(part 1 of 2)
# Autodesk Inventor assembly: 110033226_iam_04_大橋塔樓
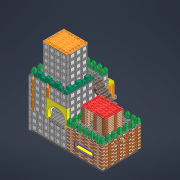
[picture p0: Inventor's stored thumbnail of the model, 180x180]
Saved by Autodesk Inventor 2022 (Build 260153000, 153)
## iProperties
Created: 2022-06-23
Part Number: 110033226_iam_04_大橋塔樓
Document SubType Name: Assembly
Designer: User
Author: User
## Documents named in this file (16)
- D:\D-disk\pomelo\大一\下學期\機械設計製圖\1100332260_LEGOproj_沒有公主城堡\110033226_iam_04_大橋塔樓.iam
- D:\D-disk\pomelo\大一\下學期\機械設計製圖\1100332260_LEGOproj_沒有公主城堡\110033226_ipt_07_磚塊樺木(2x1).ipt
- D:\D-disk\pomelo\大一\下學期\機械設計製圖\1100332260_LEGOproj_沒有公主城堡\110033226_ipt_05_房子底座.ipt
- D:\D-disk\pomelo\大一\下學期\機械設計製圖\1100332260_LEGOproj_沒有公主城堡\110033226_ipt_06_磚塊樺木(1x1).ipt
- D:\D-disk\pomelo\大一\下學期\機械設計製圖\1100332260_LEGOproj_沒有公主城堡\110033226_ipt_16_圍牆.ipt
- D:\D-disk\pomelo\大一\下學期\機械設計製圖\1100332260_LEGOproj_沒有公主城堡\110033226_ipt_08_平滑面(3x1).ipt
- D:\D-disk\pomelo\大一\下學期\機械設計製圖\1100332260_LEGOproj_沒有公主城堡\110033226_ipt_20_塔樓窗戶.ipt
- D:\D-disk\pomelo\大一\下學期\機械設計製圖\1100332260_LEGOproj_沒有公主城堡\110033226_ipt_21_柵欄.ipt
- D:\D-disk\pomelo\大一\下學期\機械設計製圖\1100332260_LEGOproj_沒有公主城堡\110033226_ipt_11_樓梯支架.ipt
- D:\D-disk\pomelo\大一\下學期\機械設計製圖\1100332260_LEGOproj_沒有公主城堡\110033226_ipt_22_塔樓牆壁.ipt
- D:\D-disk\pomelo\大一\下學期\機械設計製圖\1100332260_LEGOproj_沒有公主城堡\110033226_ipt_23_塔樓門口.ipt
- D:\D-disk\pomelo\大一\下學期\機械設計製圖\1100332260_LEGOproj_沒有公主城堡\110033226_ipt_10_木板條.ipt
- D:\D-disk\pomelo\大一\下學期\機械設計製圖\1100332260_LEGOproj_沒有公主城堡\110033226_ipt_24_直條(3x1).ipt
- D:\D-disk\pomelo\大一\下學期\機械設計製圖\1100332260_LEGOproj_沒有公主城堡\110033226_ipt_25_塔樓大窗戶.ipt
- D:\D-disk\pomelo\大一\下學期\機械設計製圖\1100332260_LEGOproj_沒有公主城堡\110033226_ipt_12_平滑面(2x1).ipt
- D:\D-disk\pomelo\大一\下學期\機械設計製圖\1100332260_LEGOproj_沒有公主城堡\110033226_ipt_18_大橋圍牆.ipt
## Components (1151 placed, 15 different names)
1. 110033226_ipt_05_房子底座:1 — 貼合:1, 貼合:2, 貼合:3, 貼合:4, 貼合:5, 貼合:13, 貼合:14, 貼合:15, 貼合:16, 貼合:17, 貼合:96, 貼合:97
2. 110033226_ipt_07_磚塊樺木(2x1):1 — 貼合:28, 貼合:29, 貼合:30, 貼合:148
3. 110033226_ipt_20_塔樓窗戶:1 — 貼合:37, 貼合:38, 貼合:39, 貼合:40
4. 110033226_ipt_20_塔樓窗戶:2 — 貼合:41, 貼合:42, 貼合:43
5. 110033226_ipt_08_平滑面(3x1):58 — 貼合:69, 貼合:70, 貼合:71, 貼合:193, 貼合:194, 貼合:195, 貼合:202, 貼合:204
6. 110033226_ipt_08_平滑面(3x1):59 — 貼合:72, 貼合:73, 貼合:74
7. 110033226_ipt_08_平滑面(3x1):60 — 貼合:75, 貼合:82, 貼合:83
8. 110033226_ipt_08_平滑面(3x1):61 — 貼合:76, 貼合:84, 貼合:85
9. 110033226_ipt_08_平滑面(3x1):62 — 貼合:78, 貼合:86, 貼合:87
10. 110033226_ipt_08_平滑面(3x1):63 — 貼合:80, 貼合:94, 貼合:95
11. 110033226_ipt_08_平滑面(3x1):64 — 貼合:77, 貼合:88, 貼合:89
12. 110033226_ipt_08_平滑面(3x1):65 — 貼合:79, 貼合:90, 貼合:91
13. 110033226_ipt_08_平滑面(3x1):66 — 貼合:81, 貼合:92, 貼合:93
14. 110033226_ipt_05_房子底座:2 — 貼合:96, 貼合:97, 貼合:98, 貼合:99, 貼合:100, 貼合:101, 對稱:1, 貼合:102, 貼合:103, 貼合:137, 貼合:138, 貼合:139, 貼合:143, 貼合:144, 貼合:145, 貼合:146, 貼合:147, 貼合:170
15. 110033226_ipt_23_塔樓門口:1 — 貼合:104, 貼合:105, 貼合:106, 貼合:179, 貼合:180, 貼合:181, 貼合:182, 貼合:183
16. 110033226_ipt_10_木板條:1 — 貼合:134, 貼合:135, 貼合:136
17. 110033226_ipt_10_木板條:33 — 貼合:128, 貼合:129, 貼合:130
18. 110033226_ipt_10_木板條:34 — 貼合:113, 貼合:114, 貼合:115, 貼合:116, 貼合:117, 貼合:118
19. 110033226_ipt_10_木板條:35 — 貼合:140, 貼合:141, 貼合:142
20. 110033226_ipt_10_木板條:36 — 貼合:131, 貼合:132, 貼合:133
21. 110033226_ipt_10_木板條:42 — 貼合:119, 貼合:120, 貼合:121
22. 110033226_ipt_24_直條(3x1):8 — 貼合:182, 貼合:183
23. 110033226_ipt_25_塔樓大窗戶:1 — 貼合:196, 貼合:197, 貼合:198
24. 110033226_ipt_16_圍牆:1 — 貼合:25, 貼合:26, 貼合:27
25. 110033226_ipt_16_圍牆:2
26. 110033226_ipt_21_柵欄:1 — 貼合:44, 貼合:45, 貼合:46, 貼合:48
27. 110033226_ipt_21_柵欄:4
28. 110033226_ipt_21_柵欄:5
29. 110033226_ipt_21_柵欄:6
30. 110033226_ipt_21_柵欄:7
31. 110033226_ipt_21_柵欄:8
32. 110033226_ipt_21_柵欄:9
33. 110033226_ipt_21_柵欄:14
34. 110033226_ipt_21_柵欄:15
35. 110033226_ipt_21_柵欄:16
36. 110033226_ipt_21_柵欄:17
37. 110033226_ipt_21_柵欄:18
38. 110033226_ipt_21_柵欄:19
39. 110033226_ipt_21_柵欄:20
40. 110033226_ipt_21_柵欄:2 — 貼合:47, 貼合:48, 貼合:49
41. 110033226_ipt_21_柵欄:10
42. 110033226_ipt_21_柵欄:11
43. 110033226_ipt_21_柵欄:12
44. 110033226_ipt_21_柵欄:13
45. 110033226_ipt_21_柵欄:21
46. 110033226_ipt_21_柵欄:22
47. 110033226_ipt_21_柵欄:23
48. 110033226_ipt_21_柵欄:24
49. 110033226_ipt_21_柵欄:25
50. 110033226_ipt_22_塔樓牆壁:2 — 對稱:1, 貼合:102, 貼合:103
51. 110033226_ipt_22_塔樓牆壁:22
52. 110033226_ipt_22_塔樓牆壁:23
53. 110033226_ipt_22_塔樓牆壁:24
54. 110033226_ipt_22_塔樓牆壁:25
55. 110033226_ipt_22_塔樓牆壁:26
56. 110033226_ipt_22_塔樓牆壁:27
57. 110033226_ipt_22_塔樓牆壁:28
58. 110033226_ipt_22_塔樓牆壁:29
59. 110033226_ipt_22_塔樓牆壁:30
60. 110033226_ipt_22_塔樓牆壁:31
61. 110033226_ipt_22_塔樓牆壁:32
62. 110033226_ipt_22_塔樓牆壁:33
63. 110033226_ipt_22_塔樓牆壁:34
64. 110033226_ipt_22_塔樓牆壁:35
65. 110033226_ipt_22_塔樓牆壁:36
66. 110033226_ipt_22_塔樓牆壁:37
67. 110033226_ipt_22_塔樓牆壁:38
68. 110033226_ipt_22_塔樓牆壁:39
69. 110033226_ipt_22_塔樓牆壁:40
70. 110033226_ipt_22_塔樓牆壁:41 — 貼合:171, 貼合:172
71. 110033226_ipt_22_塔樓牆壁:42
72. 110033226_ipt_22_塔樓牆壁:43
73. 110033226_ipt_22_塔樓牆壁:44
74. 110033226_ipt_22_塔樓牆壁:45 — 貼合:173, 貼合:174, 貼合:175
75. 110033226_ipt_22_塔樓牆壁:46 — 貼合:107, 貼合:108, 貼合:109
76. 110033226_ipt_22_塔樓牆壁:48
77. 110033226_ipt_22_塔樓牆壁:49
78. 110033226_ipt_22_塔樓牆壁:50
79. 110033226_ipt_22_塔樓牆壁:51 — 貼合:215
80. 110033226_ipt_22_塔樓牆壁:52
81. 110033226_ipt_22_塔樓牆壁:53
82. 110033226_ipt_22_塔樓牆壁:54
83. 110033226_ipt_22_塔樓牆壁:215
84. 110033226_ipt_22_塔樓牆壁:216 — 貼合:213, 貼合:214
85. 110033226_ipt_11_樓梯支架:41 — 貼合:113, 貼合:114, 貼合:118, 貼合:119, 貼合:121
86. 110033226_ipt_11_樓梯支架:42 — 貼合:120
87. 110033226_ipt_11_樓梯支架:43 — 貼合:134
88. 110033226_ipt_11_樓梯支架:44 — 貼合:135, 貼合:136
89. 110033226_ipt_11_樓梯支架:45 — 貼合:123
90. 110033226_ipt_11_樓梯支架:46 — 貼合:122, 貼合:124
91. 110033226_ipt_10_木板條:3 — 貼合:122, 貼合:123, 貼合:124
92. 110033226_ipt_10_木板條:43
93. 110033226_ipt_10_木板條:44 — 貼合:125, 貼合:126, 貼合:127
94. 110033226_ipt_11_樓梯支架:40 — 貼合:125, 貼合:126, 貼合:127, 貼合:142
95. 110033226_ipt_11_樓梯支架:47 — 貼合:140, 貼合:141
96. 110033226_ipt_11_樓梯支架:48 — 貼合:131, 貼合:133
97. 110033226_ipt_11_樓梯支架:49 — 貼合:132
98. 110033226_ipt_11_樓梯支架:50 — 貼合:129
99. 110033226_ipt_11_樓梯支架:51 — 貼合:128, 貼合:130
100. 110033226_ipt_10_木板條:39 — 貼合:137, 貼合:138, 貼合:139
101. 110033226_ipt_10_木板條:45
102. 110033226_ipt_22_塔樓牆壁:55 — 貼合:143, 貼合:144, 貼合:145, 對稱:2, 貼合:152, 貼合:153
103. 110033226_ipt_22_塔樓牆壁:140
104. 110033226_ipt_22_塔樓牆壁:141
105. 110033226_ipt_22_塔樓牆壁:142 — 貼合:196
106. 110033226_ipt_22_塔樓牆壁:143
107. 110033226_ipt_22_塔樓牆壁:144
108. 110033226_ipt_22_塔樓牆壁:145 — 貼合:149, 貼合:150, 貼合:151
109. 110033226_ipt_22_塔樓牆壁:147 — 貼合:149, 貼合:150, 貼合:151, 貼合:198
110. 110033226_ipt_22_塔樓牆壁:149
111. 110033226_ipt_22_塔樓牆壁:148 — 對稱:2, 貼合:152, 貼合:153
112. 110033226_ipt_22_塔樓牆壁:150
113. 110033226_ipt_22_塔樓牆壁:151 — 貼合:178
114. 110033226_ipt_22_塔樓牆壁:152
115. 110033226_ipt_22_塔樓牆壁:153
116. 110033226_ipt_22_塔樓牆壁:154
117. 110033226_ipt_22_塔樓牆壁:155
118. 110033226_ipt_22_塔樓牆壁:156
119. 110033226_ipt_22_塔樓牆壁:157
120. 110033226_ipt_22_塔樓牆壁:158 — 貼合:197
121. 110033226_ipt_22_塔樓牆壁:159
122. 110033226_ipt_22_塔樓牆壁:160
123. 110033226_ipt_22_塔樓牆壁:161 — 貼合:199, 貼合:200, 貼合:201
124. 110033226_ipt_22_塔樓牆壁:162 — 貼合:205
125. 110033226_ipt_07_磚塊樺木(2x1):234 — 對稱:3, 貼合:163, 貼合:164, 貼合:165, 貼合:166, 貼合:167
126. 110033226_ipt_06_磚塊樺木(1x1):234 — 貼合:165, 貼合:166, 貼合:167
127. 110033226_ipt_07_磚塊樺木(2x1):235
128. 110033226_ipt_06_磚塊樺木(1x1):235
129. 110033226_ipt_07_磚塊樺木(2x1):236
130. 110033226_ipt_06_磚塊樺木(1x1):236
131. 110033226_ipt_07_磚塊樺木(2x1):237
132. 110033226_ipt_06_磚塊樺木(1x1):237
133. 110033226_ipt_07_磚塊樺木(2x1):238
134. 110033226_ipt_06_磚塊樺木(1x1):238
135. 110033226_ipt_07_磚塊樺木(2x1):239
136. 110033226_ipt_06_磚塊樺木(1x1):239
137. 110033226_ipt_07_磚塊樺木(2x1):240
138. 110033226_ipt_06_磚塊樺木(1x1):240
139. 110033226_ipt_07_磚塊樺木(2x1):241
140. 110033226_ipt_06_磚塊樺木(1x1):241
141. 110033226_ipt_07_磚塊樺木(2x1):242
142. 110033226_ipt_06_磚塊樺木(1x1):242
143. 110033226_ipt_07_磚塊樺木(2x1):243
144. 110033226_ipt_06_磚塊樺木(1x1):243
145. 110033226_ipt_07_磚塊樺木(2x1):244
146. 110033226_ipt_06_磚塊樺木(1x1):244
147. 110033226_ipt_07_磚塊樺木(2x1):245
148. 110033226_ipt_06_磚塊樺木(1x1):245
149. 110033226_ipt_07_磚塊樺木(2x1):246
150. 110033226_ipt_06_磚塊樺木(1x1):246
151. 110033226_ipt_07_磚塊樺木(2x1):247
152. 110033226_ipt_06_磚塊樺木(1x1):247
153. 110033226_ipt_07_磚塊樺木(2x1):248
154. 110033226_ipt_06_磚塊樺木(1x1):248
155. 110033226_ipt_07_磚塊樺木(2x1):249
156. 110033226_ipt_06_磚塊樺木(1x1):249
157. 110033226_ipt_07_磚塊樺木(2x1):250
158. 110033226_ipt_06_磚塊樺木(1x1):250
159. 110033226_ipt_07_磚塊樺木(2x1):251
160. 110033226_ipt_06_磚塊樺木(1x1):251
161. 110033226_ipt_07_磚塊樺木(2x1):252
162. 110033226_ipt_06_磚塊樺木(1x1):252
163. 110033226_ipt_07_磚塊樺木(2x1):253
164. 110033226_ipt_06_磚塊樺木(1x1):253
165. 110033226_ipt_07_磚塊樺木(2x1):228 — 貼合:57, 貼合:58, 貼合:59, 貼合:61, 貼合:62
166. 110033226_ipt_06_磚塊樺木(1x1):229 — 貼合:60, 貼合:61, 貼合:62
167. 110033226_ipt_07_磚塊樺木(2x1):254
168. 110033226_ipt_06_磚塊樺木(1x1):254
169. 110033226_ipt_07_磚塊樺木(2x1):259
170. 110033226_ipt_06_磚塊樺木(1x1):259
171. 110033226_ipt_07_磚塊樺木(2x1):264
172. 110033226_ipt_06_磚塊樺木(1x1):264
173. 110033226_ipt_07_磚塊樺木(2x1):269
174. 110033226_ipt_06_磚塊樺木(1x1):269
175. 110033226_ipt_07_磚塊樺木(2x1):274
176. 110033226_ipt_06_磚塊樺木(1x1):274
177. 110033226_ipt_07_磚塊樺木(2x1):279
178. 110033226_ipt_06_磚塊樺木(1x1):279
179. 110033226_ipt_07_磚塊樺木(2x1):284
180. 110033226_ipt_06_磚塊樺木(1x1):284
181. 110033226_ipt_07_磚塊樺木(2x1):289
182. 110033226_ipt_06_磚塊樺木(1x1):289
183. 110033226_ipt_07_磚塊樺木(2x1):294
184. 110033226_ipt_06_磚塊樺木(1x1):294 — 貼合:245
185. 110033226_ipt_06_磚塊樺木(1x1):299 — 對稱:4, 貼合:168, 貼合:169
186. 110033226_ipt_06_磚塊樺木(1x1):300
187. 110033226_ipt_06_磚塊樺木(1x1):301
188. 110033226_ipt_06_磚塊樺木(1x1):302
189. 110033226_ipt_06_磚塊樺木(1x1):303
190. 110033226_ipt_06_磚塊樺木(1x1):304
191. 110033226_ipt_06_磚塊樺木(1x1):305
192. 110033226_ipt_06_磚塊樺木(1x1):306
193. 110033226_ipt_06_磚塊樺木(1x1):307
194. 110033226_ipt_06_磚塊樺木(1x1):308 — 貼合:241, 貼合:242, 貼合:243, 貼合:244
195. 110033226_ipt_24_直條(3x1):1 — 貼合:170, 貼合:171, 貼合:172
196. 110033226_ipt_24_直條(3x1):2
197. 110033226_ipt_24_直條(3x1):3
198. 110033226_ipt_24_直條(3x1):4
199. 110033226_ipt_22_塔樓牆壁:194 — 貼合:173, 貼合:174, 貼合:175
200. 110033226_ipt_22_塔樓牆壁:206
201. 110033226_ipt_22_塔樓牆壁:207
202. 110033226_ipt_22_塔樓牆壁:208 — 貼合:184
203. 110033226_ipt_22_塔樓牆壁:209 — 貼合:185, 貼合:186
204. 110033226_ipt_24_直條(3x1):5 — 貼合:176, 貼合:177, 貼合:178
205. 110033226_ipt_24_直條(3x1):6
206. 110033226_ipt_24_直條(3x1):7
207. 110033226_ipt_22_塔樓牆壁:193 — 貼合:179, 貼合:180, 貼合:181
208. 110033226_ipt_22_塔樓牆壁:210
209. 110033226_ipt_22_塔樓牆壁:211
210. 110033226_ipt_22_塔樓牆壁:212
211. 110033226_ipt_22_塔樓牆壁:213
212. 110033226_ipt_22_塔樓牆壁:214
213. 110033226_ipt_22_塔樓牆壁:217 — 貼合:184, 貼合:185, 貼合:186
214. 110033226_ipt_22_塔樓牆壁:218
215. 110033226_ipt_22_塔樓牆壁:219
216. 110033226_ipt_22_塔樓牆壁:220
217. 110033226_ipt_22_塔樓牆壁:221
218. 110033226_ipt_22_塔樓牆壁:222 — 貼合:218
219. 110033226_ipt_22_塔樓牆壁:223
220. 110033226_ipt_22_塔樓牆壁:224 — 貼合:216, 貼合:217
221. 110033226_ipt_22_塔樓牆壁:225 — 貼合:187, 貼合:188, 貼合:189
222. 110033226_ipt_22_塔樓牆壁:226 — 貼合:190, 貼合:191, 貼合:192
223. 110033226_ipt_21_柵欄:26 — 貼合:190, 貼合:191, 貼合:192
224. 110033226_ipt_21_柵欄:27
225. 110033226_ipt_21_柵欄:28
226. 110033226_ipt_21_柵欄:29
227. 110033226_ipt_21_柵欄:30
228. 110033226_ipt_21_柵欄:31
229. 110033226_ipt_21_柵欄:32
230. 110033226_ipt_21_柵欄:33
231. 110033226_ipt_21_柵欄:34
232. 110033226_ipt_21_柵欄:35
233. 110033226_ipt_21_柵欄:36
234. 110033226_ipt_21_柵欄:37
235. 110033226_ipt_08_平滑面(3x1):67 — 貼合:193, 貼合:194, 貼合:195
236. 110033226_ipt_08_平滑面(3x1):70 — 貼合:203
237. 110033226_ipt_08_平滑面(3x1):71 — 貼合:208, 貼合:222, 貼合:223, 貼合:224
238. 110033226_ipt_08_平滑面(3x1):72
239. 110033226_ipt_08_平滑面(3x1):73 — 貼合:225, 貼合:226
240. 110033226_ipt_08_平滑面(3x1):74
241. 110033226_ipt_08_平滑面(3x1):75
242. 110033226_ipt_08_平滑面(3x1):76 — 貼合:227
243. 110033226_ipt_08_平滑面(3x1):77
244. 110033226_ipt_08_平滑面(3x1):78
245. 110033226_ipt_08_平滑面(3x1):79
246. 110033226_ipt_08_平滑面(3x1):80
247. 110033226_ipt_08_平滑面(3x1):81
248. 110033226_ipt_08_平滑面(3x1):82
249. 110033226_ipt_08_平滑面(3x1):83
250. 110033226_ipt_08_平滑面(3x1):84
251. 110033226_ipt_08_平滑面(3x1):85
252. 110033226_ipt_08_平滑面(3x1):86
253. 110033226_ipt_08_平滑面(3x1):87
254. 110033226_ipt_08_平滑面(3x1):88
255. 110033226_ipt_08_平滑面(3x1):89
256. 110033226_ipt_08_平滑面(3x1):90
257. 110033226_ipt_08_平滑面(3x1):91 — 貼合:228, 貼合:229, 貼合:230
258. 110033226_ipt_08_平滑面(3x1):92
259. 110033226_ipt_08_平滑面(3x1):93
260. 110033226_ipt_08_平滑面(3x1):94
261. 110033226_ipt_08_平滑面(3x1):95 — 貼合:206
262. 110033226_ipt_08_平滑面(3x1):96
263. 110033226_ipt_08_平滑面(3x1):97
264. 110033226_ipt_08_平滑面(3x1):98 — 貼合:207
265. 110033226_ipt_22_塔樓牆壁:227 — 貼合:199, 貼合:200, 貼合:201
266. 110033226_ipt_22_塔樓牆壁:229
267. 110033226_ipt_22_塔樓牆壁:230
268. 110033226_ipt_22_塔樓牆壁:231
269. 110033226_ipt_22_塔樓牆壁:232
270. 110033226_ipt_22_塔樓牆壁:233
271. 110033226_ipt_22_塔樓牆壁:234
272. 110033226_ipt_22_塔樓牆壁:235 — 貼合:211, 貼合:212
273. 110033226_ipt_08_平滑面(3x1):100 — 貼合:202, 貼合:203, 貼合:204
274. 110033226_ipt_08_平滑面(3x1):102 — 貼合:210
275. 110033226_ipt_08_平滑面(3x1):101 — 貼合:205, 貼合:206, 貼合:207
276. 110033226_ipt_08_平滑面(3x1):103
277. 110033226_ipt_08_平滑面(3x1):104 — 貼合:209, 貼合:220
278. 110033226_ipt_08_平滑面(3x1):105
279. 110033226_ipt_08_平滑面(3x1):106
280. 110033226_ipt_08_平滑面(3x1):107
281. 110033226_ipt_12_平滑面(2x1):1 — 貼合:208, 貼合:209, 貼合:210, 貼合:219, 貼合:221
282. 110033226_ipt_12_平滑面(2x1):3
283. 110033226_ipt_21_柵欄:42 — 貼合:211, 貼合:212
284. 110033226_ipt_21_柵欄:43
285. 110033226_ipt_21_柵欄:44
286. 110033226_ipt_21_柵欄:45
287. 110033226_ipt_21_柵欄:46
288. 110033226_ipt_21_柵欄:47
289. 110033226_ipt_21_柵欄:48
290. 110033226_ipt_21_柵欄:49
291. 110033226_ipt_21_柵欄:50
292. 110033226_ipt_21_柵欄:51
293. 110033226_ipt_21_柵欄:52
294. 110033226_ipt_21_柵欄:53
295. 110033226_ipt_18_大橋圍牆:2 — 貼合:213, 貼合:214, 貼合:215
296. 110033226_ipt_18_大橋圍牆:3
297. 110033226_ipt_18_大橋圍牆:4
298. 110033226_ipt_18_大橋圍牆:1 — 貼合:216, 貼合:217, 貼合:218
299. 110033226_ipt_18_大橋圍牆:5
300. 110033226_ipt_18_大橋圍牆:6
301. 110033226_ipt_12_平滑面(2x1):4 — 貼合:234, 貼合:235, 貼合:236
302. 110033226_ipt_12_平滑面(2x1):8
303. 110033226_ipt_12_平滑面(2x1):9
304. 110033226_ipt_12_平滑面(2x1):10
305. 110033226_ipt_12_平滑面(2x1):11
306. 110033226_ipt_12_平滑面(2x1):12
307. 110033226_ipt_12_平滑面(2x1):13
308. 110033226_ipt_12_平滑面(2x1):14
309. 110033226_ipt_12_平滑面(2x1):15
310. 110033226_ipt_12_平滑面(2x1):16
311. 110033226_ipt_12_平滑面(2x1):17
312. 110033226_ipt_12_平滑面(2x1):18
313. 110033226_ipt_12_平滑面(2x1):19
314. 110033226_ipt_12_平滑面(2x1):20
315. 110033226_ipt_12_平滑面(2x1):21
316. 110033226_ipt_12_平滑面(2x1):22
317. 110033226_ipt_12_平滑面(2x1):23
318. 110033226_ipt_12_平滑面(2x1):24
319. 110033226_ipt_12_平滑面(2x1):25
320. 110033226_ipt_12_平滑面(2x1):26
321. 110033226_ipt_12_平滑面(2x1):27
322. 110033226_ipt_12_平滑面(2x1):28
323. 110033226_ipt_12_平滑面(2x1):29
324. 110033226_ipt_12_平滑面(2x1):30
325. 110033226_ipt_12_平滑面(2x1):31
326. 110033226_ipt_12_平滑面(2x1):32
327. 110033226_ipt_12_平滑面(2x1):33
328. 110033226_ipt_12_平滑面(2x1):34
329. 110033226_ipt_22_塔樓牆壁:298 — 貼合:237, 貼合:238, 貼合:239
330. 110033226_ipt_22_塔樓牆壁:299
331. 110033226_ipt_22_塔樓牆壁:300
332. 110033226_ipt_12_平滑面(2x1):35
333. 110033226_ipt_12_平滑面(2x1):36
334. 110033226_ipt_12_平滑面(2x1):37
335. 110033226_ipt_12_平滑面(2x1):38
336. 110033226_ipt_12_平滑面(2x1):39
337. 110033226_ipt_12_平滑面(2x1):40
338. 110033226_ipt_12_平滑面(2x1):41
339. 110033226_ipt_12_平滑面(2x1):42
340. 110033226_ipt_12_平滑面(2x1):43
341. 110033226_ipt_12_平滑面(2x1):44
342. 110033226_ipt_12_平滑面(2x1):45
343. 110033226_ipt_12_平滑面(2x1):46
344. 110033226_ipt_12_平滑面(2x1):47
345. 110033226_ipt_12_平滑面(2x1):48
346. 110033226_ipt_08_平滑面(3x1):110 — 貼合:240, 貼合:241, 貼合:242
347. 110033226_ipt_08_平滑面(3x1):111
348. 110033226_ipt_08_平滑面(3x1):112
349. 110033226_ipt_08_平滑面(3x1):113
350. 110033226_ipt_08_平滑面(3x1):108 — 貼合:243, 貼合:244, 貼合:245
351. 110033226_ipt_08_平滑面(3x1):114
352. 110033226_ipt_08_平滑面(3x1):115
353. 110033226_ipt_08_平滑面(3x1):116
354. 110033226_ipt_08_平滑面(3x1):117
355. 110033226_ipt_08_平滑面(3x1):118
356. 110033226_ipt_08_平滑面(3x1):119
357. 110033226_ipt_08_平滑面(3x1):120
358. 110033226_ipt_08_平滑面(3x1):121
359. 110033226_ipt_08_平滑面(3x1):122
360. 110033226_ipt_08_平滑面(3x1):123
361. 110033226_ipt_08_平滑面(3x1):124
362. 110033226_ipt_06_磚塊樺木(1x1):2 — 貼合:22, 貼合:23, 貼合:24
363. 110033226_ipt_07_磚塊樺木(2x1):2 — 貼合:19, 貼合:20, 貼合:21, 貼合:23
364. 110033226_ipt_06_磚塊樺木(1x1):1 — 貼合:16, 貼合:17, 貼合:18, 貼合:19, 貼合:21
365. 110033226_ipt_07_磚塊樺木(2x1):5 — 貼合:13, 貼合:14, 貼合:15, 貼合:18, 貼合:20, 貼合:22, 貼合:24
366. 110033226_ipt_06_磚塊樺木(1x1):60
367. 110033226_ipt_07_磚塊樺木(2x1):61
368. 110033226_ipt_06_磚塊樺木(1x1):61
369. 110033226_ipt_07_磚塊樺木(2x1):62
370. 110033226_ipt_06_磚塊樺木(1x1):62
371. 110033226_ipt_07_磚塊樺木(2x1):63
372. 110033226_ipt_06_磚塊樺木(1x1):63
373. 110033226_ipt_07_磚塊樺木(2x1):64
374. 110033226_ipt_06_磚塊樺木(1x1):64
375. 110033226_ipt_07_磚塊樺木(2x1):65
376. 110033226_ipt_06_磚塊樺木(1x1):65
377. 110033226_ipt_07_磚塊樺木(2x1):66
378. 110033226_ipt_06_磚塊樺木(1x1):66
379. 110033226_ipt_07_磚塊樺木(2x1):67
380. 110033226_ipt_06_磚塊樺木(1x1):67
381. 110033226_ipt_07_磚塊樺木(2x1):68
382. 110033226_ipt_06_磚塊樺木(1x1):68
383. 110033226_ipt_07_磚塊樺木(2x1):69
384. 110033226_ipt_06_磚塊樺木(1x1):69
385. 110033226_ipt_07_磚塊樺木(2x1):70
386. 110033226_ipt_06_磚塊樺木(1x1):70
387. 110033226_ipt_07_磚塊樺木(2x1):71
388. 110033226_ipt_06_磚塊樺木(1x1):71
389. 110033226_ipt_07_磚塊樺木(2x1):72
390. 110033226_ipt_06_磚塊樺木(1x1):72
391. 110033226_ipt_07_磚塊樺木(2x1):73
392. 110033226_ipt_06_磚塊樺木(1x1):73
393. 110033226_ipt_07_磚塊樺木(2x1):74
394. 110033226_ipt_06_磚塊樺木(1x1):74
395. 110033226_ipt_07_磚塊樺木(2x1):75
396. 110033226_ipt_06_磚塊樺木(1x1):75
397. 110033226_ipt_07_磚塊樺木(2x1):76
398. 110033226_ipt_06_磚塊樺木(1x1):76
399. 110033226_ipt_07_磚塊樺木(2x1):77
400. 110033226_ipt_06_磚塊樺木(1x1):77
401. 110033226_ipt_07_磚塊樺木(2x1):78
402. 110033226_ipt_06_磚塊樺木(1x1):78
403. 110033226_ipt_07_磚塊樺木(2x1):79
404. 110033226_ipt_06_磚塊樺木(1x1):79
405. 110033226_ipt_07_磚塊樺木(2x1):80
406. 110033226_ipt_06_磚塊樺木(1x1):80
407. 110033226_ipt_07_磚塊樺木(2x1):81
408. 110033226_ipt_06_磚塊樺木(1x1):81
409. 110033226_ipt_07_磚塊樺木(2x1):82
410. 110033226_ipt_06_磚塊樺木(1x1):82
411. 110033226_ipt_07_磚塊樺木(2x1):83
412. 110033226_ipt_06_磚塊樺木(1x1):83
413. 110033226_ipt_07_磚塊樺木(2x1):84
414. 110033226_ipt_06_磚塊樺木(1x1):84
415. 110033226_ipt_07_磚塊樺木(2x1):85
416. 110033226_ipt_06_磚塊樺木(1x1):85
417. 110033226_ipt_07_磚塊樺木(2x1):86
418. 110033226_ipt_06_磚塊樺木(1x1):86
419. 110033226_ipt_07_磚塊樺木(2x1):87
420. 110033226_ipt_06_磚塊樺木(1x1):87
421. 110033226_ipt_07_磚塊樺木(2x1):88
422. 110033226_ipt_06_磚塊樺木(1x1):88
423. 110033226_ipt_07_磚塊樺木(2x1):89
424. 110033226_ipt_06_磚塊樺木(1x1):89
425. 110033226_ipt_07_磚塊樺木(2x1):90
426. 110033226_ipt_06_磚塊樺木(1x1):90
427. 110033226_ipt_07_磚塊樺木(2x1):91
428. 110033226_ipt_06_磚塊樺木(1x1):91
429. 110033226_ipt_07_磚塊樺木(2x1):92
430. 110033226_ipt_06_磚塊樺木(1x1):92
431. 110033226_ipt_07_磚塊樺木(2x1):93
432. 110033226_ipt_06_磚塊樺木(1x1):93
433. 110033226_ipt_07_磚塊樺木(2x1):94
434. 110033226_ipt_06_磚塊樺木(1x1):94
435. 110033226_ipt_07_磚塊樺木(2x1):95
436. 110033226_ipt_06_磚塊樺木(1x1):95
437. 110033226_ipt_07_磚塊樺木(2x1):96
438. 110033226_ipt_06_磚塊樺木(1x1):96
439. 110033226_ipt_07_磚塊樺木(2x1):97
440. 110033226_ipt_06_磚塊樺木(1x1):97
441. 110033226_ipt_07_磚塊樺木(2x1):98
442. 110033226_ipt_06_磚塊樺木(1x1):98
443. 110033226_ipt_07_磚塊樺木(2x1):99
444. 110033226_ipt_06_磚塊樺木(1x1):99
445. 110033226_ipt_07_磚塊樺木(2x1):100
446. 110033226_ipt_06_磚塊樺木(1x1):104
447. 110033226_ipt_07_磚塊樺木(2x1):105
448. 110033226_ipt_06_磚塊樺木(1x1):105
449. 110033226_ipt_07_磚塊樺木(2x1):106
450. 110033226_ipt_06_磚塊樺木(1x1):106
451. 110033226_ipt_07_磚塊樺木(2x1):107
452. 110033226_ipt_06_磚塊樺木(1x1):107
453. 110033226_ipt_07_磚塊樺木(2x1):108
454. 110033226_ipt_06_磚塊樺木(1x1):108
455. 110033226_ipt_07_磚塊樺木(2x1):109
456. 110033226_ipt_06_磚塊樺木(1x1):109
457. 110033226_ipt_07_磚塊樺木(2x1):110
458. 110033226_ipt_06_磚塊樺木(1x1):110
459. 110033226_ipt_07_磚塊樺木(2x1):111
460. 110033226_ipt_06_磚塊樺木(1x1):111
461. 110033226_ipt_07_磚塊樺木(2x1):112
462. 110033226_ipt_06_磚塊樺木(1x1):112
463. 110033226_ipt_07_磚塊樺木(2x1):113
464. 110033226_ipt_06_磚塊樺木(1x1):113
465. 110033226_ipt_07_磚塊樺木(2x1):114
466. 110033226_ipt_06_磚塊樺木(1x1):114
467. 110033226_ipt_07_磚塊樺木(2x1):115
468. 110033226_ipt_06_磚塊樺木(1x1):115
469. 110033226_ipt_07_磚塊樺木(2x1):116
470. 110033226_ipt_06_磚塊樺木(1x1):116
471. 110033226_ipt_07_磚塊樺木(2x1):117
472. 110033226_ipt_06_磚塊樺木(1x1):117 — 貼合:98
473. 110033226_ipt_07_磚塊樺木(2x1):118
474. 110033226_ipt_06_磚塊樺木(1x1):118
475. 110033226_ipt_07_磚塊樺木(2x1):119
476. 110033226_ipt_06_磚塊樺木(1x1):119
477. 110033226_ipt_07_磚塊樺木(2x1):120
478. 110033226_ipt_06_磚塊樺木(1x1):120
479. 110033226_ipt_07_磚塊樺木(2x1):121
480. 110033226_ipt_06_磚塊樺木(1x1):121
481. 110033226_ipt_07_磚塊樺木(2x1):122
482. 110033226_ipt_06_磚塊樺木(1x1):122
483. 110033226_ipt_07_磚塊樺木(2x1):123
484. 110033226_ipt_06_磚塊樺木(1x1):123
485. 110033226_ipt_07_磚塊樺木(2x1):124
486. 110033226_ipt_06_磚塊樺木(1x1):124
487. 110033226_ipt_07_磚塊樺木(2x1):125
488. 110033226_ipt_06_磚塊樺木(1x1):125
489. 110033226_ipt_07_磚塊樺木(2x1):126
490. 110033226_ipt_06_磚塊樺木(1x1):126
491. 110033226_ipt_07_磚塊樺木(2x1):127
492. 110033226_ipt_06_磚塊樺木(1x1):127
493. 110033226_ipt_07_磚塊樺木(2x1):128
494. 110033226_ipt_06_磚塊樺木(1x1):128
495. 110033226_ipt_07_磚塊樺木(2x1):129
496. 110033226_ipt_06_磚塊樺木(1x1):129
497. 110033226_ipt_07_磚塊樺木(2x1):130
498. 110033226_ipt_06_磚塊樺木(1x1):130
499. 110033226_ipt_07_磚塊樺木(2x1):131
500. 110033226_ipt_06_磚塊樺木(1x1):131
501. 110033226_ipt_07_磚塊樺木(2x1):132
502. 110033226_ipt_06_磚塊樺木(1x1):132
503. 110033226_ipt_07_磚塊樺木(2x1):133
504. 110033226_ipt_06_磚塊樺木(1x1):133
505. 110033226_ipt_07_磚塊樺木(2x1):134
506. 110033226_ipt_06_磚塊樺木(1x1):134
507. 110033226_ipt_07_磚塊樺木(2x1):135
508. 110033226_ipt_06_磚塊樺木(1x1):135
509. 110033226_ipt_07_磚塊樺木(2x1):136
510. 110033226_ipt_06_磚塊樺木(1x1):136
511. 110033226_ipt_07_磚塊樺木(2x1):137
512. 110033226_ipt_06_磚塊樺木(1x1):137
513. 110033226_ipt_07_磚塊樺木(2x1):138
514. 110033226_ipt_06_磚塊樺木(1x1):138
515. 110033226_ipt_07_磚塊樺木(2x1):139
516. 110033226_ipt_06_磚塊樺木(1x1):139
517. 110033226_ipt_07_磚塊樺木(2x1):140
518. 110033226_ipt_06_磚塊樺木(1x1):140
519. 110033226_ipt_07_磚塊樺木(2x1):141
520. 110033226_ipt_06_磚塊樺木(1x1):141
521. 110033226_ipt_07_磚塊樺木(2x1):142
522. 110033226_ipt_06_磚塊樺木(1x1):142
523. 110033226_ipt_07_磚塊樺木(2x1):143
524. 110033226_ipt_06_磚塊樺木(1x1):143
525. 110033226_ipt_07_磚塊樺木(2x1):144
526. 110033226_ipt_06_磚塊樺木(1x1):144
527. 110033226_ipt_07_磚塊樺木(2x1):145
528. 110033226_ipt_06_磚塊樺木(1x1):145
529. 110033226_ipt_07_磚塊樺木(2x1):146
530. 110033226_ipt_06_磚塊樺木(1x1):146
531. 110033226_ipt_07_磚塊樺木(2x1):147
532. 110033226_ipt_06_磚塊樺木(1x1):147
533. 110033226_ipt_07_磚塊樺木(2x1):148
534. 110033226_ipt_06_磚塊樺木(1x1):148
535. 110033226_ipt_07_磚塊樺木(2x1):149
536. 110033226_ipt_06_磚塊樺木(1x1):149
537. 110033226_ipt_07_磚塊樺木(2x1):150
538. 110033226_ipt_06_磚塊樺木(1x1):150
539. 110033226_ipt_07_磚塊樺木(2x1):151
540. 110033226_ipt_06_磚塊樺木(1x1):151
541. 110033226_ipt_07_磚塊樺木(2x1):152
542. 110033226_ipt_06_磚塊樺木(1x1):152
543. 110033226_ipt_07_磚塊樺木(2x1):153
544. 110033226_ipt_06_磚塊樺木(1x1):153
545. 110033226_ipt_07_磚塊樺木(2x1):154
546. 110033226_ipt_06_磚塊樺木(1x1):154
547. 110033226_ipt_07_磚塊樺木(2x1):155
548. 110033226_ipt_06_磚塊樺木(1x1):155
549. 110033226_ipt_07_磚塊樺木(2x1):156
550. 110033226_ipt_06_磚塊樺木(1x1):160
551. 110033226_ipt_07_磚塊樺木(2x1):161
552. 110033226_ipt_06_磚塊樺木(1x1):161
553. 110033226_ipt_07_磚塊樺木(2x1):162
554. 110033226_ipt_06_磚塊樺木(1x1):162
555. 110033226_ipt_07_磚塊樺木(2x1):163 — 貼合:33
556. 110033226_ipt_06_磚塊樺木(1x1):163
557. 110033226_ipt_07_磚塊樺木(2x1):164
558. 110033226_ipt_06_磚塊樺木(1x1):164
559. 110033226_ipt_07_磚塊樺木(2x1):165 — 貼合:31
560. 110033226_ipt_06_磚塊樺木(1x1):165
561. 110033226_ipt_07_磚塊樺木(2x1):166
562. 110033226_ipt_06_磚塊樺木(1x1):166
563. 110033226_ipt_07_磚塊樺木(2x1):167
564. 110033226_ipt_06_磚塊樺木(1x1):167
565. 110033226_ipt_07_磚塊樺木(2x1):168
566. 110033226_ipt_06_磚塊樺木(1x1):168
567. 110033226_ipt_07_磚塊樺木(2x1):169 — 貼合:35
568. 110033226_ipt_06_磚塊樺木(1x1):169
569. 110033226_ipt_07_磚塊樺木(2x1):170
570. 110033226_ipt_07_磚塊樺木(2x1):3 — 貼合:7, 貼合:8, 貼合:9, 貼合:12
571. 110033226_ipt_06_磚塊樺木(1x1):4 — 貼合:10, 貼合:11, 貼合:12
572. 110033226_ipt_07_磚塊樺木(2x1):6 — 貼合:1, 貼合:2, 貼合:3, 貼合:6, 貼合:7, 貼合:8, 貼合:10, 貼合:11
573. 110033226_ipt_06_磚塊樺木(1x1):5 — 貼合:4, 貼合:5, 貼合:6, 貼合:9
574. 110033226_ipt_07_磚塊樺木(2x1):7
575. 110033226_ipt_06_磚塊樺木(1x1):6
576. 110033226_ipt_07_磚塊樺木(2x1):8
577. 110033226_ipt_06_磚塊樺木(1x1):7
578. 110033226_ipt_07_磚塊樺木(2x1):9
579. 110033226_ipt_06_磚塊樺木(1x1):8
580. 110033226_ipt_07_磚塊樺木(2x1):10
581. 110033226_ipt_06_磚塊樺木(1x1):9
582. 110033226_ipt_07_磚塊樺木(2x1):11
583. 110033226_ipt_06_磚塊樺木(1x1):10
584. 110033226_ipt_07_磚塊樺木(2x1):12
585. 110033226_ipt_06_磚塊樺木(1x1):11
586. 110033226_ipt_07_磚塊樺木(2x1):13
587. 110033226_ipt_06_磚塊樺木(1x1):12
588. 110033226_ipt_07_磚塊樺木(2x1):14
589. 110033226_ipt_06_磚塊樺木(1x1):13
590. 110033226_ipt_07_磚塊樺木(2x1):15
591. 110033226_ipt_06_磚塊樺木(1x1):14
592. 110033226_ipt_07_磚塊樺木(2x1):16
593. 110033226_ipt_06_磚塊樺木(1x1):15
594. 110033226_ipt_07_磚塊樺木(2x1):17
595. 110033226_ipt_06_磚塊樺木(1x1):16
596. 110033226_ipt_07_磚塊樺木(2x1):18
597. 110033226_ipt_06_磚塊樺木(1x1):17
598. 110033226_ipt_07_磚塊樺木(2x1):19
599. 110033226_ipt_06_磚塊樺木(1x1):18
600. 110033226_ipt_07_磚塊樺木(2x1):20
601. 110033226_ipt_06_磚塊樺木(1x1):19
602. 110033226_ipt_07_磚塊樺木(2x1):21 — 貼合:37, 貼合:40
603. 110033226_ipt_06_磚塊樺木(1x1):20
604. 110033226_ipt_07_磚塊樺木(2x1):22
605. 110033226_ipt_06_磚塊樺木(1x1):21
606. 110033226_ipt_07_磚塊樺木(2x1):27
607. 110033226_ipt_06_磚塊樺木(1x1):26
608. 110033226_ipt_07_磚塊樺木(2x1):28
609. 110033226_ipt_06_磚塊樺木(1x1):27
610. 110033226_ipt_07_磚塊樺木(2x1):29
611. 110033226_ipt_06_磚塊樺木(1x1):28
612. 110033226_ipt_07_磚塊樺木(2x1):30
613. 110033226_ipt_06_磚塊樺木(1x1):29
614. 110033226_ipt_07_磚塊樺木(2x1):31
615. 110033226_ipt_06_磚塊樺木(1x1):30
616. 110033226_ipt_07_磚塊樺木(2x1):32
617. 110033226_ipt_06_磚塊樺木(1x1):31
618. 110033226_ipt_07_磚塊樺木(2x1):33
619. 110033226_ipt_06_磚塊樺木(1x1):32
620. 110033226_ipt_07_磚塊樺木(2x1):34
621. 110033226_ipt_06_磚塊樺木(1x1):33
622. 110033226_ipt_07_磚塊樺木(2x1):35
623. 110033226_ipt_06_磚塊樺木(1x1):34
624. 110033226_ipt_07_磚塊樺木(2x1):36
625. 110033226_ipt_06_磚塊樺木(1x1):35
626. 110033226_ipt_07_磚塊樺木(2x1):41
627. 110033226_ipt_06_磚塊樺木(1x1):40
628. 110033226_ipt_07_磚塊樺木(2x1):42
629. 110033226_ipt_06_磚塊樺木(1x1):41
630. 110033226_ipt_07_磚塊樺木(2x1):43
631. 110033226_ipt_06_磚塊樺木(1x1):42
632. 110033226_ipt_07_磚塊樺木(2x1):44
633. 110033226_ipt_06_磚塊樺木(1x1):43
634. 110033226_ipt_07_磚塊樺木(2x1):45
635. 110033226_ipt_06_磚塊樺木(1x1):44
636. 110033226_ipt_07_磚塊樺木(2x1):46
637. 110033226_ipt_06_磚塊樺木(1x1):45
638. 110033226_ipt_07_磚塊樺木(2x1):47
639. 110033226_ipt_06_磚塊樺木(1x1):46
640. 110033226_ipt_07_磚塊樺木(2x1):48
641. 110033226_ipt_06_磚塊樺木(1x1):47
642. 110033226_ipt_07_磚塊樺木(2x1):49
643. 110033226_ipt_06_磚塊樺木(1x1):48
644. 110033226_ipt_07_磚塊樺木(2x1):50
645. 110033226_ipt_06_磚塊樺木(1x1):49
646. 110033226_ipt_07_磚塊樺木(2x1):51
647. 110033226_ipt_06_磚塊樺木(1x1):50 — 貼合:38
648. 110033226_ipt_07_磚塊樺木(2x1):52 — 貼合:39
649. 110033226_ipt_06_磚塊樺木(1x1):51
650. 110033226_ipt_07_磚塊樺木(2x1):53
651. 110033226_ipt_06_磚塊樺木(1x1):52
652. 110033226_ipt_07_磚塊樺木(2x1):54
653. 110033226_ipt_06_磚塊樺木(1x1):53
654. 110033226_ipt_07_磚塊樺木(2x1):55
655. 110033226_ipt_06_磚塊樺木(1x1):54
656. 110033226_ipt_07_磚塊樺木(2x1):56
657. 110033226_ipt_06_磚塊樺木(1x1):55
658. 110033226_ipt_07_磚塊樺木(2x1):57
659. 110033226_ipt_06_磚塊樺木(1x1):56
660. 110033226_ipt_07_磚塊樺木(2x1):58
661. 110033226_ipt_06_磚塊樺木(1x1):57
662. 110033226_ipt_07_磚塊樺木(2x1):59 — 貼合:32
663. 110033226_ipt_06_磚塊樺木(1x1):58
664. 110033226_ipt_07_磚塊樺木(2x1):60
665. 110033226_ipt_06_磚塊樺木(1x1):59
666. 110033226_ipt_07_磚塊樺木(2x1):171
667. 110033226_ipt_06_磚塊樺木(1x1):170
668. 110033226_ipt_07_磚塊樺木(2x1):172 — 貼合:25, 貼合:26, 貼合:27
669. 110033226_ipt_06_磚塊樺木(1x1):171
670. 110033226_ipt_07_磚塊樺木(2x1):173
671. 110033226_ipt_06_磚塊樺木(1x1):172
672. 110033226_ipt_07_磚塊樺木(2x1):174
673. 110033226_ipt_06_磚塊樺木(1x1):173
674. 110033226_ipt_07_磚塊樺木(2x1):175
675. 110033226_ipt_06_磚塊樺木(1x1):174
676. 110033226_ipt_07_磚塊樺木(2x1):176
677. 110033226_ipt_06_磚塊樺木(1x1):175 — 貼合:42
678. 110033226_ipt_07_磚塊樺木(2x1):177
679. 110033226_ipt_06_磚塊樺木(1x1):176
680. 110033226_ipt_07_磚塊樺木(2x1):178
681. 110033226_ipt_06_磚塊樺木(1x1):177
682. 110033226_ipt_07_磚塊樺木(2x1):179
683. 110033226_ipt_06_磚塊樺木(1x1):178
684. 110033226_ipt_07_磚塊樺木(2x1):180
685. 110033226_ipt_06_磚塊樺木(1x1):179
686. 110033226_ipt_07_磚塊樺木(2x1):181
687. 110033226_ipt_06_磚塊樺木(1x1):180
688. 110033226_ipt_07_磚塊樺木(2x1):182
689. 110033226_ipt_06_磚塊樺木(1x1):181
690. 110033226_ipt_07_磚塊樺木(2x1):183
691. 110033226_ipt_06_磚塊樺木(1x1):182
692. 110033226_ipt_07_磚塊樺木(2x1):184
693. 110033226_ipt_06_磚塊樺木(1x1):183
694. 110033226_ipt_07_磚塊樺木(2x1):185
695. 110033226_ipt_06_磚塊樺木(1x1):184
696. 110033226_ipt_07_磚塊樺木(2x1):186
697. 110033226_ipt_06_磚塊樺木(1x1):185
698. 110033226_ipt_07_磚塊樺木(2x1):187
699. 110033226_ipt_06_磚塊樺木(1x1):186
700. 110033226_ipt_07_磚塊樺木(2x1):188
701. 110033226_ipt_06_磚塊樺木(1x1):187
702. 110033226_ipt_07_磚塊樺木(2x1):193
703. 110033226_ipt_06_磚塊樺木(1x1):192
704. 110033226_ipt_07_磚塊樺木(2x1):194
705. 110033226_ipt_06_磚塊樺木(1x1):193
706. 110033226_ipt_07_磚塊樺木(2x1):195
707. 110033226_ipt_06_磚塊樺木(1x1):194
708. 110033226_ipt_07_磚塊樺木(2x1):196
709. 110033226_ipt_06_磚塊樺木(1x1):195
710. 110033226_ipt_07_磚塊樺木(2x1):197
711. 110033226_ipt_06_磚塊樺木(1x1):196
712. 110033226_ipt_07_磚塊樺木(2x1):198
713. 110033226_ipt_06_磚塊樺木(1x1):197
714. 110033226_ipt_07_磚塊樺木(2x1):199
715. 110033226_ipt_06_磚塊樺木(1x1):198
716. 110033226_ipt_07_磚塊樺木(2x1):200
717. 110033226_ipt_06_磚塊樺木(1x1):199
718. 110033226_ipt_07_磚塊樺木(2x1):201 — 貼合:41, 貼合:43
719. 110033226_ipt_06_磚塊樺木(1x1):200
720. 110033226_ipt_07_磚塊樺木(2x1):202
721. 110033226_ipt_06_磚塊樺木(1x1):201
722. 110033226_ipt_07_磚塊樺木(2x1):207
723. 110033226_ipt_06_磚塊樺木(1x1):206
724. 110033226_ipt_07_磚塊樺木(2x1):208
725. 110033226_ipt_06_磚塊樺木(1x1):207
726. 110033226_ipt_07_磚塊樺木(2x1):209
727. 110033226_ipt_06_磚塊樺木(1x1):208
728. 110033226_ipt_07_磚塊樺木(2x1):210
729. 110033226_ipt_06_磚塊樺木(1x1):209
730. 110033226_ipt_07_磚塊樺木(2x1):211
731. 110033226_ipt_06_磚塊樺木(1x1):210
732. 110033226_ipt_07_磚塊樺木(2x1):212
733. 110033226_ipt_06_磚塊樺木(1x1):211
734. 110033226_ipt_07_磚塊樺木(2x1):213
735. 110033226_ipt_06_磚塊樺木(1x1):212
736. 110033226_ipt_07_磚塊樺木(2x1):214 — 貼合:28, 貼合:29
737. 110033226_ipt_06_磚塊樺木(1x1):213 — 貼合:30
738. 110033226_ipt_07_磚塊樺木(2x1):215
739. 110033226_ipt_06_磚塊樺木(1x1):214
740. 110033226_ipt_07_磚塊樺木(2x1):216
741. 110033226_ipt_06_磚塊樺木(1x1):215
742. 110033226_ipt_07_磚塊樺木(2x1):217
743. 110033226_ipt_06_磚塊樺木(1x1):216
744. 110033226_ipt_07_磚塊樺木(2x1):218
745. 110033226_ipt_06_磚塊樺木(1x1):217
746. 110033226_ipt_07_磚塊樺木(2x1):219
747. 110033226_ipt_06_磚塊樺木(1x1):218
748. 110033226_ipt_07_磚塊樺木(2x1):220
749. 110033226_ipt_06_磚塊樺木(1x1):219
750. 110033226_ipt_07_磚塊樺木(2x1):221
751. 110033226_ipt_06_磚塊樺木(1x1):220
752. 110033226_ipt_07_磚塊樺木(2x1):222
753. 110033226_ipt_06_磚塊樺木(1x1):221
754. 110033226_ipt_07_磚塊樺木(2x1):223
755. 110033226_ipt_06_磚塊樺木(1x1):222
756. 110033226_ipt_07_磚塊樺木(2x1):224
757. 110033226_ipt_06_磚塊樺木(1x1):223
758. 110033226_ipt_07_磚塊樺木(2x1):225 — 貼合:34
759. 110033226_ipt_06_磚塊樺木(1x1):224 — 貼合:36
760. 110033226_ipt_07_磚塊樺木(2x1):226
761. 110033226_ipt_06_磚塊樺木(1x1):225
762. 110033226_ipt_08_平滑面(3x1):1 — 貼合:31, 貼合:32, 貼合:33
763. 110033226_ipt_08_平滑面(3x1):4
764. 110033226_ipt_08_平滑面(3x1):5
765. 110033226_ipt_08_平滑面(3x1):6
766. 110033226_ipt_08_平滑面(3x1):7
767. 110033226_ipt_08_平滑面(3x1):8
768. 110033226_ipt_08_平滑面(3x1):9
769. 110033226_ipt_08_平滑面(3x1):10
770. 110033226_ipt_08_平滑面(3x1):18
771. 110033226_ipt_08_平滑面(3x1):19
772. 110033226_ipt_08_平滑面(3x1):20
773. 110033226_ipt_08_平滑面(3x1):21
774. 110033226_ipt_08_平滑面(3x1):22
775. 110033226_ipt_08_平滑面(3x1):23 — 對稱:4, 貼合:168
776. 110033226_ipt_08_平滑面(3x1):24 — 對稱:3
777. 110033226_ipt_08_平滑面(3x1):25
778. 110033226_ipt_08_平滑面(3x1):26
779. 110033226_ipt_08_平滑面(3x1):27
780. 110033226_ipt_08_平滑面(3x1):28
781. 110033226_ipt_08_平滑面(3x1):29
782. 110033226_ipt_08_平滑面(3x1):30
783. 110033226_ipt_08_平滑面(3x1):31
784. 110033226_ipt_08_平滑面(3x1):32
785. 110033226_ipt_08_平滑面(3x1):33
786. 110033226_ipt_08_平滑面(3x1):34
787. 110033226_ipt_08_平滑面(3x1):35 — 貼合:60
788. 110033226_ipt_08_平滑面(3x1):36
789. 110033226_ipt_08_平滑面(3x1):37 — 貼合:63, 貼合:64
790. 110033226_ipt_08_平滑面(3x1):38
791. 110033226_ipt_08_平滑面(3x1):39 — 貼合:59
792. 110033226_ipt_08_平滑面(3x1):40
793. 110033226_ipt_08_平滑面(3x1):41 — 貼合:65
794. 110033226_ipt_08_平滑面(3x1):42
795. 110033226_ipt_08_平滑面(3x1):43 — 貼合:57, 貼合:58
796. 110033226_ipt_08_平滑面(3x1):44
797. 110033226_ipt_08_平滑面(3x1):45
798. 110033226_ipt_08_平滑面(3x1):46
799. 110033226_ipt_08_平滑面(3x1):47
800. 110033226_ipt_08_平滑面(3x1):48 — 貼合:50, 貼合:51, 貼合:53, 貼合:55
801. 110033226_ipt_08_平滑面(3x1):49
802. 110033226_ipt_08_平滑面(3x1):50
803. 110033226_ipt_08_平滑面(3x1):51
804. 110033226_ipt_08_平滑面(3x1):52
805. 110033226_ipt_08_平滑面(3x1):53
806. 110033226_ipt_08_平滑面(3x1):54
807. 110033226_ipt_08_平滑面(3x1):55
808. 110033226_ipt_08_平滑面(3x1):56
809. 110033226_ipt_08_平滑面(3x1):57
810. 110033226_ipt_08_平滑面(3x1):2 — 貼合:34, 貼合:35, 貼合:36
811. 110033226_ipt_08_平滑面(3x1):11
812. 110033226_ipt_08_平滑面(3x1):12 — 貼合:49
813. 110033226_ipt_08_平滑面(3x1):13 — 貼合:44, 貼合:45, 貼合:46, 貼合:47
814. 110033226_ipt_08_平滑面(3x1):14
815. 110033226_ipt_08_平滑面(3x1):15
816. 110033226_ipt_08_平滑面(3x1):16
817. 110033226_ipt_08_平滑面(3x1):17
818. 110033226_ipt_11_樓梯支架:1 — 貼合:63, 貼合:64, 貼合:65, 貼合:66, 貼合:67, 貼合:68
819. 110033226_ipt_11_樓梯支架:2 — 貼合:66, 貼合:67, 貼合:68, 貼合:81
820. 110033226_ipt_11_樓梯支架:6 — 貼合:79
821. 110033226_ipt_11_樓梯支架:7 — 貼合:77
822. 110033226_ipt_11_樓梯支架:8 — 貼合:78
823. 110033226_ipt_11_樓梯支架:9 — 貼合:85
824. 110033226_ipt_11_樓梯支架:10 — 貼合:75, 貼合:82
825. 110033226_ipt_11_樓梯支架:11
826. 110033226_ipt_11_樓梯支架:12 — 貼合:94, 貼合:95
827. 110033226_ipt_11_樓梯支架:13
828. 110033226_ipt_11_樓梯支架:14
829. 110033226_ipt_11_樓梯支架:15
830. 110033226_ipt_11_樓梯支架:16 — 貼合:86, 貼合:87
831. 110033226_ipt_11_樓梯支架:17 — 貼合:84
832. 110033226_ipt_11_樓梯支架:18 — 貼合:83
833. 110033226_ipt_11_樓梯支架:19 — 貼合:70, 貼合:74
834. 110033226_ipt_11_樓梯支架:20 — 貼合:80
835. 110033226_ipt_11_樓梯支架:21 — 貼合:92, 貼合:93
836. 110033226_ipt_11_樓梯支架:22 — 貼合:90, 貼合:91
837. 110033226_ipt_11_樓梯支架:23 — 貼合:88, 貼合:89
838. 110033226_ipt_11_樓梯支架:24
839. 110033226_ipt_11_樓梯支架:25
840. 110033226_ipt_11_樓梯支架:26
841. 110033226_ipt_11_樓梯支架:27 — 貼合:69, 貼合:71, 貼合:73
842. 110033226_ipt_11_樓梯支架:28
843. 110033226_ipt_11_樓梯支架:29
844. 110033226_ipt_11_樓梯支架:30
845. 110033226_ipt_11_樓梯支架:31
846. 110033226_ipt_11_樓梯支架:32
847. 110033226_ipt_11_樓梯支架:33 — 貼合:76
848. 110033226_ipt_11_樓梯支架:34
849. 110033226_ipt_11_樓梯支架:35 — 貼合:72
850. 110033226_ipt_22_塔樓牆壁:1 — 貼合:99, 貼合:100, 貼合:101
851. 110033226_ipt_22_塔樓牆壁:5
852. 110033226_ipt_22_塔樓牆壁:6
853. 110033226_ipt_22_塔樓牆壁:7
854. 110033226_ipt_22_塔樓牆壁:8
855. 110033226_ipt_22_塔樓牆壁:9
856. 110033226_ipt_22_塔樓牆壁:10
857. 110033226_ipt_22_塔樓牆壁:11
858. 110033226_ipt_22_塔樓牆壁:12
859. 110033226_ipt_22_塔樓牆壁:13
860. 110033226_ipt_22_塔樓牆壁:14
861. 110033226_ipt_22_塔樓牆壁:15
862. 110033226_ipt_22_塔樓牆壁:16 — 貼合:105, 貼合:110, 貼合:111, 貼合:112
863. 110033226_ipt_22_塔樓牆壁:17 — 貼合:104
864. 110033226_ipt_22_塔樓牆壁:18
865. 110033226_ipt_22_塔樓牆壁:19 — 貼合:106, 貼合:108
866. 110033226_ipt_22_塔樓牆壁:20 — 貼合:107, 貼合:109
867. 110033226_ipt_22_塔樓牆壁:21 — 貼合:176, 貼合:177
868. 110033226_ipt_22_塔樓牆壁:104 — 貼合:146, 貼合:147, 貼合:148
869. 110033226_ipt_22_塔樓牆壁:105
870. 110033226_ipt_22_塔樓牆壁:106
871. 110033226_ipt_22_塔樓牆壁:107
872. 110033226_ipt_22_塔樓牆壁:108
873. 110033226_ipt_22_塔樓牆壁:109
874. 110033226_ipt_22_塔樓牆壁:110
875. 110033226_ipt_22_塔樓牆壁:111
876. 110033226_ipt_22_塔樓牆壁:112
877. 110033226_ipt_22_塔樓牆壁:113
878. 110033226_ipt_22_塔樓牆壁:114
879. 110033226_ipt_22_塔樓牆壁:115
880. 110033226_ipt_22_塔樓牆壁:116
881. 110033226_ipt_22_塔樓牆壁:117
882. 110033226_ipt_22_塔樓牆壁:118
883. 110033226_ipt_22_塔樓牆壁:119
884. 110033226_ipt_22_塔樓牆壁:120
885. 110033226_ipt_22_塔樓牆壁:121
886. 110033226_ipt_22_塔樓牆壁:122
887. 110033226_ipt_22_塔樓牆壁:123
888. 110033226_ipt_22_塔樓牆壁:124
889. 110033226_ipt_22_塔樓牆壁:125
890. 110033226_ipt_22_塔樓牆壁:126
891. 110033226_ipt_22_塔樓牆壁:127
892. 110033226_ipt_22_塔樓牆壁:128
893. 110033226_ipt_22_塔樓牆壁:129 — 貼合:154, 貼合:155
894. 110033226_ipt_22_塔樓牆壁:130
895. 110033226_ipt_22_塔樓牆壁:131
896. 110033226_ipt_22_塔樓牆壁:132
897. 110033226_ipt_22_塔樓牆壁:133
898. 110033226_ipt_22_塔樓牆壁:134
899. 110033226_ipt_22_塔樓牆壁:135 — 貼合:156, 貼合:157, 貼合:158
900. 110033226_ipt_22_塔樓牆壁:136
901. 110033226_ipt_22_塔樓牆壁:137 — 貼合:159
902. 110033226_ipt_22_塔樓牆壁:138
903. 110033226_ipt_22_塔樓牆壁:139
904. 110033226_ipt_22_塔樓牆壁:146 — 貼合:157, 貼合:158, 貼合:159
905. 110033226_ipt_22_塔樓牆壁:163
906. 110033226_ipt_22_塔樓牆壁:164
907. 110033226_ipt_22_塔樓牆壁:165
908. 110033226_ipt_22_塔樓牆壁:166
909. 110033226_ipt_22_塔樓牆壁:167
910. 110033226_ipt_22_塔樓牆壁:168
911. 110033226_ipt_22_塔樓牆壁:169
912. 110033226_ipt_22_塔樓牆壁:170
913. 110033226_ipt_22_塔樓牆壁:171
914. 110033226_ipt_22_塔樓牆壁:172
915. 110033226_ipt_22_塔樓牆壁:173
916. 110033226_ipt_22_塔樓牆壁:174
917. 110033226_ipt_22_塔樓牆壁:175
918. 110033226_ipt_22_塔樓牆壁:176
919. 110033226_ipt_22_塔樓牆壁:177
920. 110033226_ipt_22_塔樓牆壁:178
921. 110033226_ipt_22_塔樓牆壁:179
922. 110033226_ipt_22_塔樓牆壁:180
923. 110033226_ipt_22_塔樓牆壁:181
924. 110033226_ipt_22_塔樓牆壁:182
925. 110033226_ipt_22_塔樓牆壁:183
926. 110033226_ipt_22_塔樓牆壁:184
927. 110033226_ipt_22_塔樓牆壁:185
928. 110033226_ipt_22_塔樓牆壁:186
929. 110033226_ipt_22_塔樓牆壁:187
930. 110033226_ipt_22_塔樓牆壁:188
931. 110033226_ipt_22_塔樓牆壁:189
932. 110033226_ipt_22_塔樓牆壁:190
933. 110033226_ipt_22_塔樓牆壁:191
934. 110033226_ipt_22_塔樓牆壁:192 — 貼合:160, 貼合:161, 貼合:162
935. 110033226_ipt_22_塔樓牆壁:195
936. 110033226_ipt_22_塔樓牆壁:196
937. 110033226_ipt_22_塔樓牆壁:197
938. 110033226_ipt_22_塔樓牆壁:198
939. 110033226_ipt_22_塔樓牆壁:199
940. 110033226_ipt_22_塔樓牆壁:200
941. 110033226_ipt_22_塔樓牆壁:201
942. 110033226_ipt_22_塔樓牆壁:202
943. 110033226_ipt_22_塔樓牆壁:203
944. 110033226_ipt_22_塔樓牆壁:204
945. 110033226_ipt_22_塔樓牆壁:205
946. 110033226_ipt_10_木板條:2 — 貼合:110, 貼合:111, 貼合:112
947. 110033226_ipt_10_木板條:4
948. 110033226_ipt_10_木板條:5
949. 110033226_ipt_10_木板條:6
950. 110033226_ipt_10_木板條:7
951. 110033226_ipt_10_木板條:8
952. 110033226_ipt_10_木板條:9
953. 110033226_ipt_10_木板條:10
954. 110033226_ipt_10_木板條:11
955. 110033226_ipt_10_木板條:12
956. 110033226_ipt_10_木板條:13
957. 110033226_ipt_10_木板條:14
958. 110033226_ipt_10_木板條:15
959. 110033226_ipt_10_木板條:16
960. 110033226_ipt_10_木板條:17
961. 110033226_ipt_10_木板條:18
962. 110033226_ipt_10_木板條:19
963. 110033226_ipt_10_木板條:20
964. 110033226_ipt_10_木板條:21
965. 110033226_ipt_10_木板條:22
966. 110033226_ipt_10_木板條:23
967. 110033226_ipt_10_木板條:24
968. 110033226_ipt_10_木板條:25
969. 110033226_ipt_10_木板條:26
970. 110033226_ipt_10_木板條:27
971. 110033226_ipt_10_木板條:28
972. 110033226_ipt_10_木板條:29 — 貼合:117
973. 110033226_ipt_10_木板條:30 — 貼合:115
974. 110033226_ipt_10_木板條:31 — 貼合:116
975. 110033226_ipt_10_木板條:32
976. 110033226_ipt_10_木板條:46
977. 110033226_ipt_10_木板條:47
978. 110033226_ipt_10_木板條:48
979. 110033226_ipt_10_木板條:49
980. 110033226_ipt_10_木板條:50